# Autodesk Inventor assembly: ReleaseAssembly
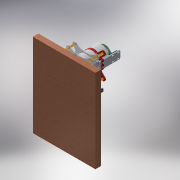
[picture p0: Inventor's stored thumbnail of the model, 180x180]
Saved by Autodesk Inventor 2018.2 (Build 222227000, 227)
## iProperties
Created: 2018-03-27
Part Number: ReleaseAssembly
Document SubType Name: Assembly
Designer: mansu
Author: mansu
## Documents named in this file (6)
- C:\Users\Moochster\OneDrive\Documents\2018 UBC\ELEC 391\Controller\cad\release\ReleaseAssembly.iam
- C:\Users\Moochster\OneDrive\Documents\2018 UBC\ELEC 391\Controller\cad\release\PitchAssembly.iam
- C:\Users\Moochster\OneDrive\Documents\2018 UBC\ELEC 391\Controller\cad\release\YawAssembly.iam
- C:\Users\Moochster\OneDrive\Documents\2018 UBC\ELEC 391\Controller\cad\release\WoodBase.ipt
- C:\Users\Moochster\OneDrive\Documents\2018 UBC\ELEC 391\Controller\cad\release\pcb.iam
- C:\Users\Moochster\OneDrive\Documents\2018 UBC\ELEC 391\Controller\cad\release\Fasteners\StandoffM4x5B.ipt
## Components (8 placed, 5 different names)
1. PitchAssembly:1 [sub-assembly] — Flush:1, Mate:2
2. YawAssembly:1 [sub-assembly] — Mate:1, Flush:1
3. WoodBase:1 — Mate:2, Mate:3
4. pcb:1 [sub-assembly] — Insert:1, Insert:2, Insert:3, Insert:4
5. StandoffM4x5B:1 — Insert:3, Mate:3
6. StandoffM4x5B:2 — Insert:1
7. StandoffM4x5B:3 — Insert:4
8. StandoffM4x5B:4 — Insert:2
## Relationships (8: Insert 4, Mate 3, Flush 1)
- Mate:1: YawAssembly:1
- Flush:1: PitchAssembly:1 ↔ YawAssembly:1
- Mate:2: PitchAssembly:1 ↔ WoodBase:1
- Insert:1: pcb:1 ↔ StandoffM4x5B:2
- Insert:2: pcb:1 ↔ StandoffM4x5B:4
- Insert:3: pcb:1 ↔ StandoffM4x5B:1
- Insert:4: pcb:1 ↔ StandoffM4x5B:3
- Mate:3: WoodBase:1 ↔ StandoffM4x5B:1
